# Autodesk Inventor assembly: Right Front Wheel with hub shaft and pulley
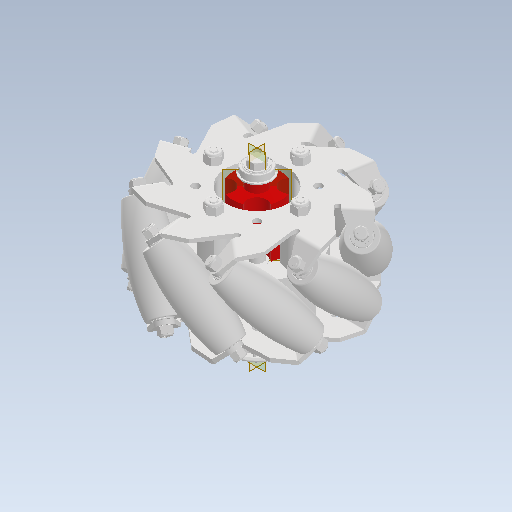
[picture p0: Inventor's stored thumbnail of the model, 512x512]
Saved by Autodesk Inventor 2020 (Build 240168000, 168)
## iProperties
Created: 2020-02-22
Part Number: Right Front Wheel with hub shaft and pulley
Document SubType Name: Assembly
Designer: ball
Author: ball
## Documents named in this file (7)
- D:\FTC8863\2019 Robot\Mecanum Drive Train Metal\Right Front Wheel with hub shaft and pulley.iam
- D:\FTC8863\2019 Robot\Mecanum Drive Train Metal\Right Front Wheel with hub.iam
- D:\FTC8863\GoBilda\2102 Parts\2102-0008-0090.ipt
- D:\FTC8863\GoBilda\3414 Parts\3414-4008-0016 assembly.iam
- D:\FTC8863\GoBilda\1601 Parts\1601-0014-0008.ipt
- D:\FTC8863\GoBilda\2807 Parts\2807-0811-0500.ipt
- D:\FTC8863\2019 Robot\Mecanum Drive Train Metal\wheel spacer for bearing.ipt
## Components (7 placed, 6 different names)
1. Right Front Wheel with hub:1 [sub-assembly] — Mate:1, Mate:2, Mate:3, Mate:12
2. 2102-0008-0090:1 — Mate:1, Mate:2, Mate:4, Mate:5, Mate:6, Mate:7, Mate:9, Flush:1, Angle:1, Mate:11
3. 3414-4008-0016 assembly:1 [sub-assembly] — Mate:3, Mate:4, Mate:5, Mate:8
4. 1601-0014-0008:1 — Mate:6, Mate:13
5. 1601-0014-0008:2 — Mate:7, Mate:10, Flush:1
6. 2807-0811-0500:1 — Mate:8, Mate:9, Mate:10
7. wheel spacer for bearing:1 — Angle:1, Mate:11, Mate:12, Mate:13
## Relationships (15: Mate 13, Flush 1, Angle 1)
- Mate:1: Right Front Wheel with hub:1 ↔ 2102-0008-0090:1
- Mate:2: Right Front Wheel with hub:1 ↔ 2102-0008-0090:1
- Mate:3: Right Front Wheel with hub:1 ↔ 3414-4008-0016 assembly:1
- Mate:4: 2102-0008-0090:1 ↔ 3414-4008-0016 assembly:1
- Mate:5: 2102-0008-0090:1 ↔ 3414-4008-0016 assembly:1
- Mate:6: 2102-0008-0090:1 ↔ 1601-0014-0008:1
- Mate:7: 2102-0008-0090:1 ↔ 1601-0014-0008:2
- Mate:8: 3414-4008-0016 assembly:1 ↔ 2807-0811-0500:1
- Mate:9: 2102-0008-0090:1 ↔ 2807-0811-0500:1
- Mate:10: 1601-0014-0008:2 ↔ 2807-0811-0500:1
- Flush:1 (-6.1595 mm): 2102-0008-0090:1 ↔ 1601-0014-0008:2
- Angle:1 (45 deg): 2102-0008-0090:1 ↔ wheel spacer for bearing:1
- Mate:11: 2102-0008-0090:1 ↔ wheel spacer for bearing:1
- Mate:12: Right Front Wheel with hub:1 ↔ wheel spacer for bearing:1
- Mate:13: 1601-0014-0008:1 ↔ wheel spacer for bearing:1
